# Autodesk Inventor assembly: SAR330
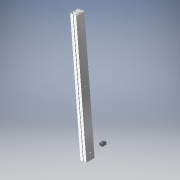
[picture p0: Inventor's stored thumbnail of the model, 180x180]
Saved by Autodesk Inventor 2019 (Build 230136000, 136)
## iProperties
Category: PARTsolutions
Company: MISUMI
Created: 2019-04-19
Part Number: SAR330
Catalog Web Link: www.cadenas.de
Description: SAR3-Slide Rails - Aluminum Alloy - Three-Step Slide Rails
Vendor: MISUMI
Document SubType Name: Assembly
Designer: psadmin
Manufacturer: MISUMI
Mass: 180.874 g
Surface Area: 598.523 cm^2
Volume: 66.9905 cm^3
Density: 2.7 g/cm^3
PSOL_IDENT_0: {$CADENAS_DATA\23d-libs\misumi\metric\07_slide_rails\sar3_asmtab.prj},168 {VTYP=3D},{STYP=ASSTAB},{N
PSOL_IDENT_1: B=SAR330},{LINA=SAR330},{NN=SAR3},{DATE=30.03.2018 01:39:43},{GEOMDATE=01.03.2017 00:48:28},{VERSION=
PSOL_IDENT_2: },{LINEID=10},{WBVAR=NO},{WBNUMERIC=NO}  {NB=SAR330},{LINA=SAR330},{KT=DUMMY},{PN=SAR330},{TP=SAR3},
PSOL_IDENT_3: {TYPE=SAR3},{MAT1=Aluminum Alloy},{ST1=Clear Anodizing},{MAT2=Aluminum Alloy},{ST2=Clear Anodizing},
PSOL_IDENT_4: {MAT3=Steel},{NO=30},{RL=300},{TD=345},{A=135},{B=270},{C=135},{D=270},{RLO=147},{PPATH=sar3_series\
PSOL_IDENT_5: \sar3_templ.prj}
NN: SAR3
NT: Slide Rails - Aluminum Alloy - Three-Step Slide Rails
NB: SAR330
NBSYN: $PN.
LINA: SAR330
PN: SAR330
TP: SAR3
MAT1: Aluminum Alloy
ST1: Clear Anodizing
MAT2: Aluminum Alloy
ST2: Clear Anodizing
MAT3: Steel
NO: 30
RL: 300
TD: 345
A: 135
B: 270
C: 135
D: 270
RLO: 147
SUPPLIER: MISUMI
ARTICLENO: SAR330
BOMINFO: SAR330
CREATOR: CADENAS GmbH
Title: SAR330
Author: Cadenas PARTsolutions
Comments: Slide Rails - Aluminum Alloy - Three-Step Slide Rails
## Documents named in this file (5)
- C:\Robotics\CAD\COTSParts\Misumi_Slides\AIS2018\SAR330.iam
- C:\Robotics\CAD\COTSParts\Misumi_Slides\AIS2018\SAR330-30_r.ipt
- C:\Robotics\CAD\COTSParts\Misumi_Slides\AIS2018\SAR330-30_b.ipt
- C:\Robotics\CAD\COTSParts\Misumi_Slides\AIS2018\SAR330_ba.ipt
- C:\Robotics\CAD\2019-20_CAD\offseason\random ideas\end peice for slides.ipt
## Components (8 placed, 4 different names)
1. SAR330-30_r:1 — Tangent:1, Tangent:2, Tangent:3, Tangent:4, Tangent:5, Tangent:6, Tangent:7, Tangent:8, Tangent:16, Tangent:17, Tangent:18, Tangent:19, Tangent:20, Tangent:21, Tangent:22, Tangent:23
2. SAR330-30_b:1 — Tangent:9, Tangent:11, Tangent:15, Tangent:24, Tangent:25, Tangent:29, Tangent:31
3. SAR330-30_b:2 — Tangent:10, Tangent:12, Tangent:13, Tangent:14, Tangent:26, Tangent:27, Tangent:28, Tangent:30
4. SAR330_ba:1 — Tangent:4, Tangent:8, Tangent:12, Tangent:14, Tangent:20, Tangent:21, Tangent:27, Tangent:30
5. SAR330_ba:2 — Tangent:1, Tangent:6, Tangent:10, Tangent:13, Tangent:16, Tangent:17, Tangent:26, Tangent:28
6. SAR330_ba:3 — Tangent:2, Tangent:5, Tangent:9, Tangent:18, Tangent:19, Tangent:24, Tangent:29
7. SAR330_ba:4 — Tangent:3, Tangent:7, Tangent:11, Tangent:15, Tangent:22, Tangent:23, Tangent:25, Tangent:31
8. end peice for slides:1
## Relationships (31: Tangent 31)
- Tangent:1: SAR330-30_r:1 ↔ SAR330_ba:2
- Tangent:2: SAR330-30_r:1 ↔ SAR330_ba:3
- Tangent:3: SAR330-30_r:1 ↔ SAR330_ba:4
- Tangent:4: SAR330-30_r:1 ↔ SAR330_ba:1
- Tangent:5: SAR330-30_r:1 ↔ SAR330_ba:3
- Tangent:6: SAR330-30_r:1 ↔ SAR330_ba:2
- Tangent:7: SAR330-30_r:1 ↔ SAR330_ba:4
- Tangent:8: SAR330-30_r:1 ↔ SAR330_ba:1
- Tangent:9: SAR330-30_b:1 ↔ SAR330_ba:3
- Tangent:10: SAR330-30_b:2 ↔ SAR330_ba:2
- Tangent:11: SAR330-30_b:1 ↔ SAR330_ba:4
- Tangent:12: SAR330-30_b:2 ↔ SAR330_ba:1
- Tangent:13: SAR330-30_b:2 ↔ SAR330_ba:2
- Tangent:14: SAR330-30_b:2 ↔ SAR330_ba:1
- Tangent:15: SAR330-30_b:1 ↔ SAR330_ba:4
- Tangent:16: SAR330-30_r:1 ↔ SAR330_ba:2
- Tangent:17: SAR330-30_r:1 ↔ SAR330_ba:2
- Tangent:18: SAR330-30_r:1 ↔ SAR330_ba:3
- Tangent:19: SAR330-30_r:1 ↔ SAR330_ba:3
- Tangent:20: SAR330-30_r:1 ↔ SAR330_ba:1
- Tangent:21: SAR330-30_r:1 ↔ SAR330_ba:1
- Tangent:22: SAR330-30_r:1 ↔ SAR330_ba:4
- Tangent:23: SAR330-30_r:1 ↔ SAR330_ba:4
- Tangent:24: SAR330-30_b:1 ↔ SAR330_ba:3
- Tangent:25: SAR330-30_b:1 ↔ SAR330_ba:4
- Tangent:26: SAR330-30_b:2 ↔ SAR330_ba:2
- Tangent:27: SAR330-30_b:2 ↔ SAR330_ba:1
- Tangent:28: SAR330-30_b:2 ↔ SAR330_ba:2
- Tangent:29: SAR330-30_b:1 ↔ SAR330_ba:3
- Tangent:30: SAR330-30_b:2 ↔ SAR330_ba:1
- Tangent:31: SAR330-30_b:1 ↔ SAR330_ba:4
